# Autodesk Inventor assembly: frame_3d_asm
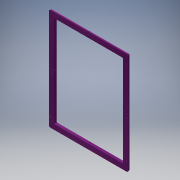
[picture p0: Inventor's stored thumbnail of the model, 180x180]
Saved by Autodesk Inventor 2017 (Build 210142000, 142)
## iProperties
Part Number: frame_3d_asm
Material: Ogólny
Document SubType Name: Assembly
Designer: Peter
Author: Peter
## Documents named in this file (3)
- F:\Workspace\Inventor\Ti\CAD\model\frame_3d_asm.iam
- F:\Workspace\Inventor\Ti\CAD\model\frame_upper_3d_1.ipt
- F:\Workspace\Inventor\Ti\CAD\model\frame_upper_3d_2.ipt
## Components (4 placed, 2 different names)
1. frame_upper_3d_1:1 — Równoległy:1, Zestawiający:1, Równoległy:2, Równoległy:6
2. frame_upper_3d_2:1 — Równoległy:1, Zestawiający:1, Równoległy:2, Zestawiający:3, Równoległy:5
3. frame_upper_3d_1:2 — Zestawiający:3
4. frame_upper_3d_2:2 — Równoległy:5, Równoległy:6
## Relationships (9: Flush 6, Mate 3)
- Równoległy:1 [Flush]: frame_upper_3d_1:1 ↔ frame_upper_3d_2:1
- Zestawiający:1 [Mate] (0.8 mm): frame_upper_3d_1:1 ↔ frame_upper_3d_2:1
- Równoległy:2 [Flush]: frame_upper_3d_1:1 ↔ frame_upper_3d_2:1
- [Flush]: frame_upper_3d_1:2 ↔ frame_upper_3d_2:2
- [Mate] (0.8 mm): frame_upper_3d_1:2 ↔ frame_upper_3d_2:2
- [Flush]: frame_upper_3d_1:2 ↔ frame_upper_3d_2:2
- Zestawiający:3 [Mate] (0.8 mm): frame_upper_3d_2:1 ↔ frame_upper_3d_1:2
- Równoległy:5 [Flush]: frame_upper_3d_2:1 ↔ frame_upper_3d_2:2
- Równoległy:6 [Flush]: frame_upper_3d_1:1 ↔ frame_upper_3d_2:2
## Named parameters: d4_d1 = 0 mm, d5_d2 = 0.8 mm, d6_d3 = 0 mm
